# Autodesk Inventor assembly: TestAssm
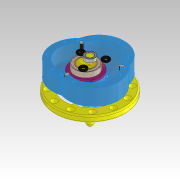
[picture p0: Inventor's stored thumbnail of the model, 180x180]
Saved by Autodesk Inventor 2020 (Build 240168000, 168)
## iProperties
Created: 2021-05-17
Part Number: TestAssm
Document SubType Name: Assembly
Designer: DDeGo
Author: DDeGo
## Documents named in this file (19)
- C:\Users\DDeGo\Documents\Drew\Projects\AirWankelEngine\cad\LiquidPiston V1.5ish\TestAssm.iam
- C:\Users\DDeGo\Documents\Drew\Projects\AirWankelEngine\cad\LiquidPiston V1.5ish\Housing.ipt
- C:\Users\DDeGo\Documents\Drew\Projects\AirWankelEngine\cad\LiquidPiston V1.5ish\Rotor.ipt
- C:\Users\DDeGo\Documents\Drew\Projects\AirWankelEngine\cad\LiquidPiston V1.5ish\CamThing.ipt
- C:\Users\DDeGo\Documents\Drew\Projects\AirWankelEngine\cad\LiquidPiston V1.5ish\TestAssm\Design Accelerator\Spur Gears1.iam
- C:\Users\DDeGo\Documents\Drew\Projects\AirWankelEngine\cad\hardware\6701 bearing.ipt
- C:\Users\DDeGo\Documents\Drew\Projects\AirWankelEngine\cad\LiquidPiston V1.5ish\Head.ipt
- C:\Users\DDeGo\Documents\Drew\Projects\AirWankelEngine\cad\LiquidPiston V1.5ish\ApexSeal.ipt
- C:\Users\DDeGo\Documents\Drew\Projects\AirWankelEngine\cad\hardware\MR85 bearing.ipt
- C:\Users\DDeGo\Documents\Drew\Projects\AirWankelEngine\cad\LiquidPiston V1.5ish\RotorTeeth.ipt
- C:\Users\DDeGo\Documents\Drew\Projects\AirWankelEngine\cad\LiquidPiston V1.5ish\Flywheel.ipt
- C:\Users\DDeGo\Documents\Drew\Projects\AirWankelEngine\cad\hardware\2x22 pin.ipt
- C:\Users\DDeGo\Documents\Drew\Projects\AirWankelEngine\cad\LiquidPiston V1.5ish\FlywheelXL.ipt
- C:\Users\DDeGo\Documents\Drew\Projects\AirWankelEngine\cad\LiquidPiston V1.5ish\MotorTestBracket.ipt
- C:\Users\DDeGo\Documents\Drew\Projects\AirWankelEngine\cad\LiquidPiston V1.5ish\2020 Extrusion.ipt
- C:\Users\DDeGo\Documents\Drew\Projects\AirWankelEngine\cad\LiquidPiston V1.5ish\TestLever.ipt
- C:\Users\DDeGo\Documents\Drew\Projects\AirWankelEngine\cad\LiquidPiston V1.5ish\TestEncoderBracket.ipt
- C:\Users\DDeGo\Documents\Drew\Projects\AirWankelEngine\cad\LiquidPiston V1.5ish\TestEncoder.ipt
- C:\Users\DDeGo\Documents\Drew\Projects\AirWankelEngine\cad\hardware\oring_2x6.ipt
## Components (23 placed, 18 different names)
1. Housing:1 — Mate:11, Mate:14, Mate:15, Mate:20, Mate:21, Mate:66, Mate:67, Mate:68, Mate:69, Mate:80, Mate:81, Flush:7, Mate:108
2. CamThing:1 — Mate:47, Flush:6, Mate:94, Mate:98, Mate:104, Rotation:1
3. Spur Gears:1 [sub-assembly]
4. 6701 bearing:1 — Flush:6, Mate:96, Mate:104, Mate:105, Mate:106, Mate:107
5. ApexSeal:1 — Mate:11, Mate:67
6. ApexSeal:2 — Mate:14, Mate:68
7. ApexSeal:3 — Mate:15, Mate:66
8. MR85 bearing:1 — Mate:20, Mate:21, Mate:32, Mate:33
9. MR85 bearing:2 — Mate:64, Mate:95, Mate:98
10. RotorTeeth:1 — Mate:96, Mate:107, Angle:1
11. Flywheel:1 — Mate:32, Mate:33, Mate:45, Mate:47, Mate:77, Mate:79
12. 2x22 pin:1 — Mate:45, Mate:78, Mate:94
13. Head:1 — Mate:64, Mate:69, Mate:95, Mate:100, Mate:101, Mate:102, Tangent:1, Tangent:2, Tangent:3, Mate:103
14. FlywheelXL:1 — Mate:77, Mate:78, Mate:79, Mate:83, Mate:84, Mate:93, Angle:2
15. MotorTestBracket:1 — Mate:80, Mate:81, Flush:7, Mate:82, Flush:8, Flush:9, Mate:103
16. 2020 Extrusion:1 — Mate:82, Flush:8, Flush:9, Mate:89, Flush:10
17. TestLever:1 — Mate:83, Mate:84
18. TestEncoderBracket:1 — Mate:89, Flush:10, Mate:90, Mate:91, Mate:92
19. TestEncoder:1 — Mate:90, Mate:91, Mate:92, Mate:93
20. oring_2x6:1 — Mate:101, Tangent:1
21. oring_2x6:2 — Mate:100, Tangent:3
22. oring_2x6:3 — Mate:102, Tangent:2
23. Rotor:2 — Mate:105, Mate:106, Angle:1, Mate:108, Rotation:1
## Relationships (51: Mate 40, Flush 5, Tangent 3, Angle 2, RelateRotation 1)
- Mate:11 (0.1 mm): Housing:1 ↔ ApexSeal:1
- Mate:14 (0.1 mm): Housing:1 ↔ ApexSeal:2
- Mate:15 (0.1 mm): Housing:1 ↔ ApexSeal:3
- Mate:20: Housing:1 ↔ MR85 bearing:1
- Mate:21: Housing:1 ↔ MR85 bearing:1
- Mate:32: MR85 bearing:1 ↔ Flywheel:1
- Mate:33: MR85 bearing:1 ↔ Flywheel:1
- Mate:45: Flywheel:1 ↔ 2x22 pin:1
- Mate:47: CamThing:1 ↔ Flywheel:1
- Flush:6: CamThing:1 ↔ 6701 bearing:1
- Mate:64: MR85 bearing:2 ↔ Head:1
- Mate:66: Housing:1 ↔ ApexSeal:3
- Mate:67: Housing:1 ↔ ApexSeal:1
- Mate:68: Housing:1 ↔ ApexSeal:2
- Mate:69 (0.2 mm): Housing:1 ↔ Head:1
- Mate:77: Flywheel:1 ↔ FlywheelXL:1
- Mate:78: 2x22 pin:1 ↔ FlywheelXL:1
- Mate:79: Flywheel:1 ↔ FlywheelXL:1
- Mate:80: Housing:1 ↔ MotorTestBracket:1
- Mate:81: Housing:1 ↔ MotorTestBracket:1
- Flush:7 (-1 mm): Housing:1 ↔ MotorTestBracket:1
- Mate:82: MotorTestBracket:1 ↔ 2020 Extrusion:1
- Flush:8: MotorTestBracket:1 ↔ 2020 Extrusion:1
- Flush:9 (5 mm): MotorTestBracket:1 ↔ 2020 Extrusion:1
- Mate:83: FlywheelXL:1 ↔ TestLever:1
- Mate:84: FlywheelXL:1 ↔ TestLever:1
- Mate:89: 2020 Extrusion:1 ↔ TestEncoderBracket:1
- Flush:10: 2020 Extrusion:1 ↔ TestEncoderBracket:1
- Mate:90: TestEncoderBracket:1 ↔ TestEncoder:1
- Mate:91: TestEncoderBracket:1 ↔ TestEncoder:1
- Mate:92: TestEncoderBracket:1 ↔ TestEncoder:1
- Mate:93: FlywheelXL:1 ↔ TestEncoder:1
- Mate:94: CamThing:1 ↔ 2x22 pin:1
- Mate:95: MR85 bearing:2 ↔ Head:1
- Mate:96: 6701 bearing:1 ↔ RotorTeeth:1
- Mate:98: CamThing:1 ↔ MR85 bearing:2
- Mate:100: Head:1 ↔ oring_2x6:2
- Mate:101: Head:1 ↔ oring_2x6:1
- Mate:102: Head:1 ↔ oring_2x6:3
- Tangent:1: Head:1 ↔ oring_2x6:1
- Tangent:2: Head:1 ↔ oring_2x6:3
- Tangent:3: Head:1 ↔ oring_2x6:2
- Mate:103: Head:1 ↔ MotorTestBracket:1
- Mate:104: CamThing:1 ↔ 6701 bearing:1
- Mate:105: 6701 bearing:1 ↔ Rotor:2
- Mate:106: 6701 bearing:1 ↔ Rotor:2
- Mate:107: 6701 bearing:1 ↔ RotorTeeth:1
- Angle:1 (0 deg): RotorTeeth:1 ↔ Rotor:2
- Mate:108 (0.5 mm): Housing:1 ↔ Rotor:2
- Rotation:1 [RelateRotation] (0.5 ul): CamThing:1 ↔ Rotor:2
- Angle:2 (0 deg): FlywheelXL:1
